# Autodesk Inventor assembly: Montagem5
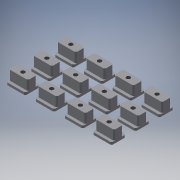
[picture p0: Inventor's stored thumbnail of the model, 180x180]
Saved by Autodesk Inventor 2018 (Build 220112000, 112)
## iProperties
Created: 2018-08-28
Part Number: Montagem5
Material: Genérico
Document SubType Name: Assembly
Designer: Georgines
Author: Georgines
## Documents named in this file (2)
- C:\Users\Georgines\Documents\EstacaoBGA\Peças 3D\Usinagem\Montagem5.iam
- C:\Users\Georgines\Documents\EstacaoBGA\Peças 3D\Usinagem\Montagem4.iam
## Components (4 placed, 1 different names)
1. Montagem4:1 [sub-assembly] — Coincidência:1, Alinhamento:1, Alinhamento:2
2. Montagem4:2 [sub-assembly] — Coincidência:1, Coincidência:2, Alinhamento:1, Alinhamento:2, Coincidência:3, Alinhamento:3, Alinhamento:4
3. Montagem4:3 [sub-assembly] — Coincidência:2, Coincidência:3, Alinhamento:3, Alinhamento:4, Alinhamento:5, Alinhamento:6, Coincidência:4
4. Montagem4:4 [sub-assembly] — Alinhamento:5, Alinhamento:6, Coincidência:4
## Relationships (10: Flush 6, Mate 4)
- Coincidência:1 [Mate] (8 mm): Montagem4:1 ↔ Montagem4:2
- Coincidência:2 [Mate] (8 mm): Montagem4:2 ↔ Montagem4:3
- Alinhamento:1 [Flush]: Montagem4:1 ↔ Montagem4:2
- Alinhamento:2 [Flush]: Montagem4:1 ↔ Montagem4:2
- Coincidência:3 [Mate] (8 mm): Montagem4:2 ↔ Montagem4:3
- Alinhamento:3 [Flush]: Montagem4:2 ↔ Montagem4:3
- Alinhamento:4 [Flush]: Montagem4:2 ↔ Montagem4:3
- Alinhamento:5 [Flush]: Montagem4:3 ↔ Montagem4:4
- Alinhamento:6 [Flush]: Montagem4:3 ↔ Montagem4:4
- Coincidência:4 [Mate] (8 mm): Montagem4:3 ↔ Montagem4:4
